# Autodesk Inventor assembly: motor_wheel_assembly
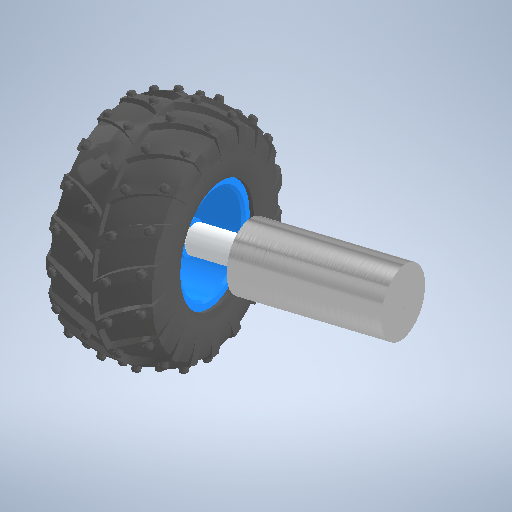
[picture p0: Inventor's stored thumbnail of the model, 512x512]
Saved by Autodesk Inventor 2025.3 (Build 293356030, 356C)
## iProperties
Created: 2026-06-28
Part Number: motor_wheel_assembly
Document SubType Name: Assembly
Designer: user
Author: user
## Documents named in this file (4)
- C:\Docs\shcool\dojo\Design_3\motor_wheel\motor_wheel_1.iam
- C:\Docs\shcool\dojo\Design_3\motor_wheel\Hub-12-Eixo6_aluminio.ipt
- C:\Docs\shcool\dojo\Design_3\motor_wheel\motor_dummy.ipt
- C:\Docs\shcool\dojo\Design_3\motor_wheel\Spiked Rubber Wheel 120mm.ipt
## Components (3 placed, 3 different names)
1. Hub-12-Eixo6_aluminio:1 — Mate:1, Mate:2, Insert:1
2. motor_dummy:1 — Insert:1
3. Spiked Rubber Wheel 120mm:1 — Mate:1, Mate:2
## Relationships (3: Mate 2, Insert 1)
- Mate:1: Hub-12-Eixo6_aluminio:1 ↔ Spiked Rubber Wheel 120mm:1
- Mate:2: Hub-12-Eixo6_aluminio:1 ↔ Spiked Rubber Wheel 120mm:1
- Insert:1: Hub-12-Eixo6_aluminio:1 ↔ motor_dummy:1
